# Autodesk Inventor assembly: Weapon (Motor-Side Pulley)
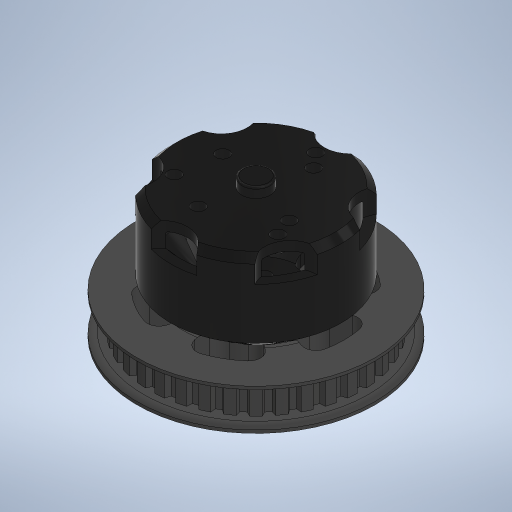
[picture p0: Inventor's stored thumbnail of the model, 512x512]
Saved by Autodesk Inventor 2023.1 (Build 271208000, 208)
## iProperties
Created: 2022-05-21
Part Number: Weapon (Motor-Side Pulley)
Document SubType Name: Assembly
Designer: Nathan Cai
Mass: 163.794 g
Surface Area: 513.523 cm^2
Volume: 53.858 cm^3
Density: 3.04123 g/cm^3
Author: Nathan Cai
## Documents named in this file (3)
- E:\Documents\Inventor\0.3rd Lawette - V3.4\Weapon (Motor-Side Pulley).iam
- E:\Documents\Inventor\0.3rd Lawette - V3.4\XL Pulley 36T .375in Wd.ipt
- E:\Documents\Inventor\0.3rd Lawette - V3.4\AeroSky_MC4822-390KV.ipt
## Components (2 placed, 2 different names)
1. XL Pulley 36T .375in Wd:1 — Mate:2, Mate:3, Mate:4
2. AeroSky_MC4822-390KV:1 — Mate:2, Mate:3, Mate:4
## Relationships (3: Mate 3)
- Mate:2 (-34.925 mm): XL Pulley 36T .375in Wd:1 ↔ AeroSky_MC4822-390KV:1
- Mate:3: XL Pulley 36T .375in Wd:1 ↔ AeroSky_MC4822-390KV:1
- Mate:4: XL Pulley 36T .375in Wd:1 ↔ AeroSky_MC4822-390KV:1
